# Autodesk Inventor assembly: Tensioner3
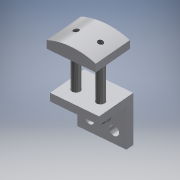
[picture p0: Inventor's stored thumbnail of the model, 180x180]
Saved by Autodesk Inventor 2017 (Build 210142000, 142)
## iProperties
Created: 2018-04-06
Part Number: Tensioner3
Document SubType Name: Assembly
Designer: User
Mass: 3.61508 g
Surface Area: 32.5533 cm^2
Volume: 3.61508 cm^3
Density: 1 g/cm^3
Author: User
## Documents named in this file (4)
- C:\Robotics\CAD\2018-19_CAD\Offseason\Tensioner3.iam
- C:\Robotics\CAD\COTSParts\Fasteners\92012A506_.125D.75L_ALLOY STEEL PRECISION SHOULDER SCREW.ipt
- C:\Robotics\CAD\2018-19_CAD\Offseason\TensionerPlate3.ipt
- C:\Robotics\CAD\2018-19_CAD\Offseason\TensionerPusher3.ipt
## Components (4 placed, 3 different names)
1. 92012A506_.125D.75L_ALLOY STEEL PRECISION SHOULDER SCREW:1 — Insert:1, Insert:4
2. 92012A506_.125D.75L_ALLOY STEEL PRECISION SHOULDER SCREW:2 — Insert:2, Insert:3
3. TensionerPlate3:1 — Insert:1, Insert:2
4. TensionerPusher3:1 — Insert:3, Insert:4
## Relationships (4: Insert 4)
- Insert:1: 92012A506_.125D.75L_ALLOY STEEL PRECISION SHOULDER SCREW:1 ↔ TensionerPlate3:1
- Insert:2: 92012A506_.125D.75L_ALLOY STEEL PRECISION SHOULDER SCREW:2 ↔ TensionerPlate3:1
- Insert:3: 92012A506_.125D.75L_ALLOY STEEL PRECISION SHOULDER SCREW:2 ↔ TensionerPusher3:1
- Insert:4: 92012A506_.125D.75L_ALLOY STEEL PRECISION SHOULDER SCREW:1 ↔ TensionerPusher3:1
